# Autodesk Inventor assembly: assembly of mach
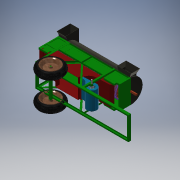
[picture p0: Inventor's stored thumbnail of the model, 180x180]
Saved by Autodesk Inventor 2017 (Build 210142000, 142)
## iProperties
Created: 2017-04-20
Part Number: assembly of mach
Document SubType Name: Assembly
Designer: master
Author: master
## Documents named in this file (9)
- C:\Users\master\Documents\Inventor\threshing machine\assembly of mach.iam
- C:\Users\master\Documents\Inventor\threshing machine\MAIN FRAME.ipt
- C:\Users\master\Documents\Inventor\threshing machine\shaker.ipt
- C:\Users\master\Documents\Inventor\threshing machine\cover.ipt
- C:\Users\master\Documents\Inventor\threshing machine\ROLLER.ipt
- C:\Users\master\Documents\Inventor\threshing machine\con-cover.ipt
- C:\Users\master\Documents\Inventor\threshing machine\blower.ipt
- C:\Users\master\Documents\Inventor\threshing machine\fan.ipt
- C:\Users\master\Documents\Inventor\threshing machine\tyre-st3.ipt
## Components (9 placed, 8 different names)
1. MAIN FRAME:1 — Mate:3, Mate:4, Mate:5, Mate:6, Mate:7, Mate:13, Flush:1, Mate:15, Mate:16, Mate:17, Mate:18, Mate:19, Mate:20, Mate:21
2. cover:1 — Mate:3, Mate:4, Flush:1
3. ROLLER:1 — Mate:5, Mate:12
4. shaker:1 — Mate:6, Mate:7
5. con-cover:1 — Mate:12, Mate:13
6. blower:1 — Mate:14, Flush:2, Mate:16
7. fan:1 — Mate:14, Flush:2, Mate:15, Mate:17
8. tyre-st3:1 — Mate:18, Mate:19
9. tyre-st3:2 — Mate:20, Mate:21
## Relationships (17: Mate 15, Flush 2)
- Mate:3: MAIN FRAME:1 ↔ cover:1
- Mate:4: MAIN FRAME:1 ↔ cover:1
- Mate:5: MAIN FRAME:1 ↔ ROLLER:1
- Mate:6: MAIN FRAME:1 ↔ shaker:1
- Mate:7: MAIN FRAME:1 ↔ shaker:1
- Mate:12: ROLLER:1 ↔ con-cover:1
- Mate:13: MAIN FRAME:1 ↔ con-cover:1
- Flush:1: MAIN FRAME:1 ↔ cover:1
- Mate:14: blower:1 ↔ fan:1
- Flush:2 (1.4 mm): blower:1 ↔ fan:1
- Mate:15: MAIN FRAME:1 ↔ fan:1
- Mate:16 (1.3 mm): MAIN FRAME:1 ↔ blower:1
- Mate:17: MAIN FRAME:1 ↔ fan:1
- Mate:18: MAIN FRAME:1 ↔ tyre-st3:1
- Mate:19: MAIN FRAME:1 ↔ tyre-st3:1
- Mate:20: MAIN FRAME:1 ↔ tyre-st3:2
- Mate:21: MAIN FRAME:1 ↔ tyre-st3:2
